# Autodesk Inventor assembly: car_finale_1_10
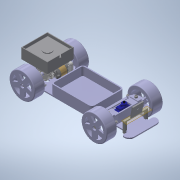
[picture p0: Inventor's stored thumbnail of the model, 180x180]
Saved by Autodesk Inventor 2020.2 (Build 242310000, 310)
## iProperties
Created: 2019-10-16
Part Number: car_finale_1_10
Material: Générique
Document SubType Name: Assembly
Designer: ropertth
Source: UnKnown
Author: ropertth
## Documents named in this file (28)
- C:\Users\anton\OneDrive\Bureau\S3_Atelier_CNC\Correction\car_inventor\car_finale_1_10.iam
- C:\Users\anton\OneDrive\Bureau\S3_Atelier_CNC\Correction\car_inventor\chassis.ipt
- C:\Users\anton\OneDrive\Bureau\S3_Atelier_CNC\Correction\car_inventor\support_arriere.ipt
- C:\Users\anton\OneDrive\Bureau\S3_Atelier_CNC\Correction\car_inventor\6661K11.ipt
- C:\Users\anton\OneDrive\Bureau\S3_Atelier_CNC\Correction\car_inventor\support_moteur_Brushless_A2212 v1.ipt
- C:\Users\anton\OneDrive\Bureau\S3_Atelier_CNC\Correction\car_inventor\NOSILEC MOT.ipt
- C:\Users\anton\OneDrive\Bureau\S3_Atelier_CNC\Correction\car_inventor\moteur_Brushless_A2212 v1.ipt
- C:\Users\anton\OneDrive\Bureau\S3_Atelier_CNC\Correction\car_inventor\arbre_arriere.ipt
- C:\Users\anton\OneDrive\Bureau\S3_Atelier_CNC\Correction\car_inventor\ecrou_roue.ipt
- C:\Users\anton\OneDrive\Bureau\S3_Atelier_CNC\Correction\car_inventor\roue_equipee.ipt
- C:\Users\anton\OneDrive\Bureau\S3_Atelier_CNC\Correction\car_inventor\goupille_2mm.ipt
- C:\Users\anton\OneDrive\Bureau\S3_Atelier_CNC\Correction\car_inventor\Engrenages cylindriques1.iam
- C:\Users\anton\OneDrive\Bureau\S3_Atelier_CNC\Correction\car_inventor\entretoise_16.ipt
- C:\Users\anton\OneDrive\Bureau\S3_Atelier_CNC\Correction\car_inventor\entretoise_43.2.ipt
- C:\Users\anton\OneDrive\Bureau\S3_Atelier_CNC\Correction\car_inventor\chassis_direction.ipt
- C:\Users\anton\OneDrive\Bureau\S3_Atelier_CNC\Correction\car_inventor\train_avant_droit.iam
- C:\Users\anton\OneDrive\Bureau\S3_Atelier_CNC\Correction\car_inventor\train_avant_gauche.iam
- C:\Users\anton\OneDrive\Bureau\S3_Atelier_CNC\Correction\car_inventor\barre_direction.ipt
- C:\Users\anton\OneDrive\Bureau\S3_Atelier_CNC\Correction\car_inventor\MicroServo9g v1_1.ipt
- C:\Users\anton\OneDrive\Bureau\S3_Atelier_CNC\Correction\car_inventor\M3x10.ipt
- C:\Users\anton\OneDrive\Bureau\S3_Atelier_CNC\Correction\car_inventor\ecrou_m3.ipt
- C:\Users\anton\OneDrive\Bureau\S3_Atelier_CNC\Correction\car_inventor\vis chc ISO4762 - M4 x 35.ipt
- C:\Users\anton\OneDrive\Bureau\S3_Atelier_CNC\Correction\car_inventor\ecrou-M4.ipt
- C:\Users\anton\OneDrive\Bureau\S3_Atelier_CNC\Correction\car_inventor\boitier_central.ipt
- C:\Users\anton\OneDrive\Bureau\Projet ROS CAO\support tige voiture.ipt
- C:\Users\anton\OneDrive\Bureau\Projet ROS CAO\tige GPS.ipt
- C:\Users\anton\OneDrive\Bureau\Projet ROS CAO\support tige gps.ipt
- C:\Users\anton\OneDrive\Bureau\Projet ROS CAO\support_caméra.ipt
## Components (68 placed, 68 different names)
1. chassis.1 — Placage:2, Placage:3, Placage:8, Placage:9, Placage:10
2. support_arriere.1
3. support_arriere.2
4. 6661K11.1
5. 6661K11.2
6. support_moteur_Brushless_A2212 v1.1
7. NOSILEC MOT.1
8. moteur_Brushless_A2212 v1.1
9. arbre_arriere.1
10. ecrou_roue.1
11. roue_equipee.1
12. goupille_2mm.1
13. ecrou_roue.2
14. roue_equipee.2
15. goupille_2mm.2
16. Engrenages cylindriques1.1 [sub-assembly]
17. entretoise_16.1
18. entretoise_43.2.1
19. entretoise_16.2
20. entretoise_16.3
21. chassis_direction.1
22. train_avant_droit.1 [sub-assembly]
23. train_avant_gauche.1 [sub-assembly]
24. barre_direction.1
25. MicroServo9g v1_1.1
26. M3x10.1
27. ecrou_m3.1
28. M3x10.2
29. M3x10.3
30. M3x10.4
31. ecrou_m3.2
32. ecrou_m3.3
33. ecrou_m3.4
34. M3x10.5
35. ecrou_m3.5
36. M3x10.6
37. ecrou_m3.6
38. ISO 4762 - M4 x 35.1
39. ecrou-M4.1
40. ISO 4762 - M4 x 35.2
41. ecrou-M4.2
42. boitier_central.1
43. M3x10.7
44. M3x10.8
45. M3x10.9
46. M3x10.10
47. ecrou_m3.7
48. ecrou_m3.8
49. ecrou_m3.9
50. ecrou_m3.10
51. M3x10.11
52. M3x10.12
53. ecrou_m3.11
54. ecrou_m3.12
55. M3x10.13
56. M3x10.14
57. M3x10.15
58. M3x10.16
59. ecrou_m3.13
60. ecrou_m3.14
61. ecrou_m3.15
62. ecrou_m3.16
63. ecrou-M4.3
64. ecrou-M4.4
65. support tige voiture:1 — Placage:2, Placage:3, Placage:4, Placage:5, Placage:8, Affleurement:1
66. tige GPS:1 — Placage:4, Placage:5, Placage:6, Placage:7
67. support tige gps:1 — Placage:6, Placage:7, Affleurement:1
68. support_caméra:1 — Placage:9, Placage:10
## Relationships (10: Mate 9, Flush 1)
- Placage:2 [Mate]: chassis.1 ↔ support tige voiture:1
- Placage:3 [Mate]: chassis.1 ↔ support tige voiture:1
- Placage:4 [Mate]: support tige voiture:1 ↔ tige GPS:1
- Placage:5 [Mate]: support tige voiture:1 ↔ tige GPS:1
- Placage:6 [Mate]: tige GPS:1 ↔ support tige gps:1
- Placage:7 [Mate]: tige GPS:1 ↔ support tige gps:1
- Placage:8 [Mate]: chassis.1 ↔ support tige voiture:1
- Affleurement:1 [Flush] (12.5 mm): support tige voiture:1 ↔ support tige gps:1
- Placage:9 [Mate]: chassis.1 ↔ support_caméra:1
- Placage:10 [Mate]: chassis.1 ↔ support_caméra:1
